# Autodesk Inventor assembly: SmallCardBox
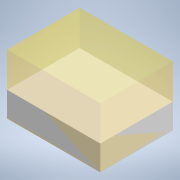
[picture p0: Inventor's stored thumbnail of the model, 180x180]
Saved by Autodesk Inventor 2022.2 (Build 262287010, 287A)
## iProperties
Created: 2022-07-12
Part Number: SmallCardBox
Document SubType Name: Assembly
Designer: keaton
Author: keaton
## Documents named in this file (2)
- C:\Users\keaton\Documents\3D Printing\KamigamiBox\SmallCardBox.iam
- C:\Users\keaton\Documents\3D Printing\KamigamiBox\BottomPlate.ipt
## Components (1 placed, 1 different names)
1. BottomPlate:1
## Named parameters: test = 25.4 mm
